# Autodesk Inventor assembly: ASY table wheel 1
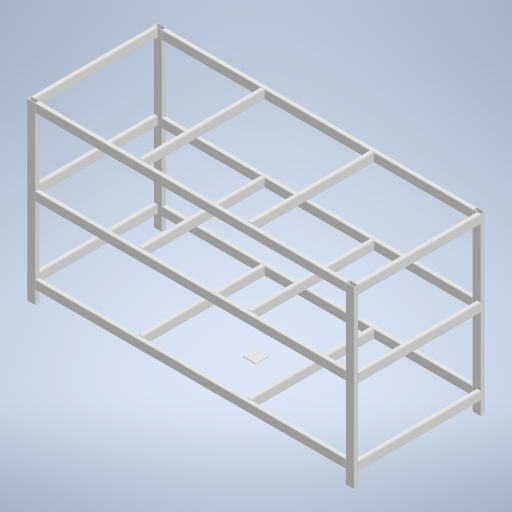
[picture p0: Inventor's stored thumbnail of the model, 512x512]
Saved by Autodesk Inventor 2023.1 (Build 271208000, 208)
## iProperties
Created: 2023-08-25
Part Number: ASY table wheel 1
Document SubType Name: Assembly
Designer: admin
_SolveAssemblyDoc: Frame Generator Solve Assembly
_Version: 25.0.0
Author: admin
## Documents named in this file (4)
- C:\Users\admin\My Drive (bigstupidbeast@gmail.com)\Inventor\Workshop\Table wheel\ASY table wheel 1.iam
- C:\Users\admin\My Drive (bigstupidbeast@gmail.com)\Inventor\Workshop\Table wheel\SKETCH roller conveyor 1.ipt
- C:\Users\admin\My Drive (bigstupidbeast@gmail.com)\Inventor\Workshop\Table wheel\Frame 1692965611507.iam
- C:\Users\admin\My Drive (bigstupidbeast@gmail.com)\Inventor\Workshop\Table wheel\plate wheel 1.ipt
## Components (3 placed, 3 different names)
1. SKETCH roller conveyor 1:1
2. Frame 1692965611507:1 [sub-assembly]
3. plate wheel 1:1 — Flush:1
## Relationships (1: Flush 1)
- Flush:1: plate wheel 1:1
